# Autodesk Inventor assembly: Assembly1
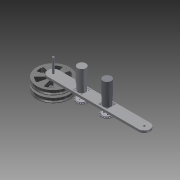
[picture p0: Inventor's stored thumbnail of the model, 180x180]
Saved by Autodesk Inventor 2011 (Build 150239000, 239)
## iProperties
Created: 2010-04-19
Part Number: Assembly1
Document SubType Name: Assembly
Designer: lucio
Author: lucio
## Documents named in this file (7)
- C:\Users\lucio\Documents\Inventor\caterpillar\Assembly1.iam
- C:\Users\lucio\Documents\Inventor\caterpillar\base side.ipt
- C:\Users\lucio\Documents\Inventor\caterpillar\mr85vel 2 etapas.ipt
- C:\Users\lucio\Documents\Inventor\caterpillar\back axle.ipt
- C:\Users\lucio\Documents\Inventor\caterpillar\back wheel.iam
- C:\Users\lucio\Documents\Inventor\caterpillar\sprocket.ipt
- C:\Users\lucio\Documents\Inventor\caterpillar\mr85vel 3 etapas.ipt
## Components (7 placed, 6 different names)
1. base side:1 — Mate:6, Mate:7, Mate:8, Mate:10, Mate:11, Mate:12, Mate:13, Mate:14
2. mr85vel 2 etapas:1 — Mate:5, Flush:1, Mate:6, Mate:7, Mate:8
3. back axle:1 — Mate:9, Flush:2, Mate:11
4. back wheel:1 [sub-assembly] — Mate:9, Flush:2, Mate:10
5. sprocket:1 — Mate:5, Flush:1
6. mr85vel 3 etapas:1 — Mate:12, Mate:13, Mate:14, Mate:15, Flush:3
7. sprocket:2 — Mate:15, Flush:3
## Relationships (14: Mate 11, Flush 3)
- Mate:5: mr85vel 2 etapas:1 ↔ sprocket:1
- Flush:1: mr85vel 2 etapas:1 ↔ sprocket:1
- Mate:6: base side:1 ↔ mr85vel 2 etapas:1
- Mate:7: base side:1 ↔ mr85vel 2 etapas:1
- Mate:8: base side:1 ↔ mr85vel 2 etapas:1
- Mate:9: back axle:1 ↔ back wheel:1
- Flush:2: back axle:1 ↔ back wheel:1
- Mate:10 (2.5 mm): base side:1 ↔ back wheel:1
- Mate:11: base side:1 ↔ back axle:1
- Mate:12: base side:1 ↔ mr85vel 3 etapas:1
- Mate:13: base side:1 ↔ mr85vel 3 etapas:1
- Mate:14: base side:1 ↔ mr85vel 3 etapas:1
- Mate:15: mr85vel 3 etapas:1 ↔ sprocket:2
- Flush:3: mr85vel 3 etapas:1 ↔ sprocket:2
